# Autodesk Inventor assembly: PojazdTrojkolowy
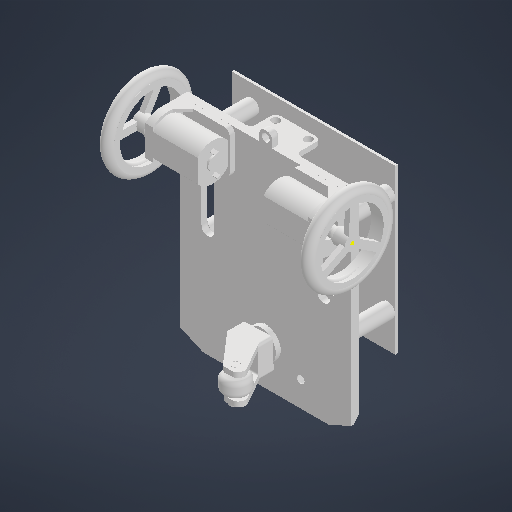
[picture p0: Inventor's stored thumbnail of the model, 512x512]
Saved by Autodesk Inventor 2026 (Build 300175000, 175)
## iProperties
Created: 2025-05-01
Part Number: PojazdTrojkolowy
Document SubType Name: Assembly
Designer: isan
Author: isan
## Documents named in this file (12)
- E:\Conan II enhanced\PojazdTrojkolowy.iam
- E:\Conan II enhanced\PodstawaTrojkolowa.ipt
- E:\Conan II enhanced\PrzegubDolny.ipt
- E:\Conan II enhanced\PrzegubGorny.ipt
- E:\Conan II enhanced\Kolek.ipt
- E:\Conan II enhanced\KolekNaKolo.ipt
- E:\Conan II enhanced\KoloPrzegubu.ipt
- E:\Conan II enhanced\Trzymak2.ipt
- E:\Conan II enhanced\Silnik.ipt
- E:\Conan II enhanced\Koło.ipt
- E:\Conan II enhanced\PCB.ipt
- E:\Conan II enhanced\Opona.ipt
## Components (15 placed, 11 different names)
1. PodstawaTrojkolowa:1 — Mate:1, Mate:2, Flush:1, Mate:3, Flush:2, Mate:4, Mate:5, Mate:6, Mate:7, Mate:26, Mate:27, Mate:28, Mate:29
2. PrzegubDolny:1 — Mate:8, Mate:9, Mate:10, Mate:11, Mate:12, Mate:13, Mate:15
3. PrzegubGorny:1 — Mate:5, Mate:6, Mate:7, Mate:8, Mate:9
4. Kolek:1 — Mate:10, Mate:11
5. KolekNaKolo:1 — Mate:12, Mate:13, Mate:14
6. KoloPrzegubu:1 — Mate:14, Mate:15
7. Trzymak2:1 — Mate:1, Flush:1, Mate:3, Mate:16, Mate:17, Mate:18
8. Trzymak2:2 — Mate:2, Flush:2, Mate:4, Mate:19, Mate:20, Mate:21
9. Silnik:1 — Mate:16, Mate:17, Mate:18, Mate:22, Mate:23
10. Silnik:2 — Mate:19, Mate:20, Mate:21, Mate:24, Mate:25
11. Koło:1 — Mate:24, Mate:25
12. Koło:2 — Mate:22, Mate:23
13. PCB:1 — Mate:26, Mate:27, Mate:28, Mate:29
14. Opona:1
15. Opona:2
## Relationships (31: Mate 29, Flush 2)
- Mate:1: PodstawaTrojkolowa:1 ↔ Trzymak2:1
- Mate:2: PodstawaTrojkolowa:1 ↔ Trzymak2:2
- Flush:1: PodstawaTrojkolowa:1 ↔ Trzymak2:1
- Mate:3 (0.1 mm): PodstawaTrojkolowa:1 ↔ Trzymak2:1
- Flush:2: PodstawaTrojkolowa:1 ↔ Trzymak2:2
- Mate:4 (0.1 mm): PodstawaTrojkolowa:1 ↔ Trzymak2:2
- Mate:5: PodstawaTrojkolowa:1 ↔ PrzegubGorny:1
- Mate:6 (0.1 mm): PodstawaTrojkolowa:1 ↔ PrzegubGorny:1
- Mate:7: PodstawaTrojkolowa:1 ↔ PrzegubGorny:1
- Mate:8: PrzegubDolny:1 ↔ PrzegubGorny:1
- Mate:9: PrzegubDolny:1 ↔ PrzegubGorny:1
- Mate:10: PrzegubDolny:1 ↔ Kolek:1
- Mate:11 (0.4 mm): PrzegubDolny:1 ↔ Kolek:1
- Mate:12: PrzegubDolny:1 ↔ KolekNaKolo:1
- Mate:13: PrzegubDolny:1 ↔ KolekNaKolo:1
- Mate:14: KolekNaKolo:1 ↔ KoloPrzegubu:1
- Mate:15 (0.2 mm): PrzegubDolny:1 ↔ KoloPrzegubu:1
- Mate:16: Trzymak2:1 ↔ Silnik:1
- Mate:17: Trzymak2:1 ↔ Silnik:1
- Mate:18: Trzymak2:1 ↔ Silnik:1
- Mate:19: Trzymak2:2 ↔ Silnik:2
- Mate:20: Trzymak2:2 ↔ Silnik:2
- Mate:21: Trzymak2:2 ↔ Silnik:2
- Mate:22: Silnik:1 ↔ Koło:2
- Mate:23: Silnik:1 ↔ Koło:2
- Mate:24: Silnik:2 ↔ Koło:1
- Mate:25: Silnik:2 ↔ Koło:1
- Mate:26: PodstawaTrojkolowa:1 ↔ PCB:1
- Mate:27: PodstawaTrojkolowa:1 ↔ PCB:1
- Mate:28: PodstawaTrojkolowa:1 ↔ PCB:1
- Mate:29: PodstawaTrojkolowa:1 ↔ PCB:1
